# Autodesk Inventor assembly: Knobass
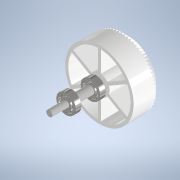
[picture p0: Inventor's stored thumbnail of the model, 180x180]
Saved by Autodesk Inventor 2022 (Build 260153000, 153)
## iProperties
Created: 2023-08-31
Part Number: Knobass
Document SubType Name: Assembly
Designer: THK
Author: THK
## Documents named in this file (6)
- C:\Users\THK\Documents\Inventor\etchasketch\Knobass.iam
- C:\Users\THK\Documents\Inventor\etchasketch\knob.ipt
- C:\Users\THK\Documents\Inventor\etchasketch\Part4.ipt
- C:\Users\THK\Documents\Inventor\Content Center Files\R2022\en-US\BS 290 SKF(30)\BS 290 SKF - SKF 626.ipt
- C:\Users\THK\Documents\Inventor\etchasketch\3mmSpacer.ipt
- C:\Users\THK\Documents\Inventor\etchasketch\18mmSpacer.ipt
## Components (6 placed, 5 different names)
1. knob:1 — Flush:1, Mate:5
2. Part4:1 — Flush:1, Mate:1, Mate:2, Mate:3, Mate:4
3. BS 290 SKF 626:1 — Mate:1, Mate:8
4. BS 290 SKF 626:2 — Mate:2, Mate:6, Mate:7
5. 3mmSpacer:1 — Mate:4, Mate:5, Mate:6
6. 18mmSpacer:1 — Mate:3, Mate:7, Mate:8
## Relationships (9: Mate 8, Flush 1)
- Flush:1: knob:1 ↔ Part4:1
- Mate:1: Part4:1 ↔ BS 290 SKF 626:1
- Mate:2: Part4:1 ↔ BS 290 SKF 626:2
- Mate:3: Part4:1 ↔ 18mmSpacer:1
- Mate:4: Part4:1 ↔ 3mmSpacer:1
- Mate:5: knob:1 ↔ 3mmSpacer:1
- Mate:6: BS 290 SKF 626:2 ↔ 3mmSpacer:1
- Mate:7: BS 290 SKF 626:2 ↔ 18mmSpacer:1
- Mate:8: BS 290 SKF 626:1 ↔ 18mmSpacer:1
